# Autodesk Inventor assembly: 垃圾桶
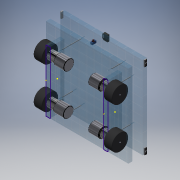
[picture p0: Inventor's stored thumbnail of the model, 180x180]
Saved by Autodesk Inventor 2017 (Build 210142000, 142)
## iProperties
Part Number: 垃圾桶
Material: 常规
Document SubType Name: Assembly
Designer: PANDA
Author: PANDA
## Documents named in this file (9)
- D:\PANDA\Study\VG100\P2\草图\垃圾桶底座.iam
- D:\PANDA\Study\VG100\P2\草图\垃圾桶底板.ipt
- D:\PANDA\Study\VG100\P2\草图\圆柱.ipt
- D:\PANDA\Study\VG100\P2\草图\马达安装板.ipt
- D:\PANDA\Study\VG100\P2\草图\轮子.ipt
- D:\PANDA\Study\VG100\P2\草图\马达.ipt
- D:\PANDA\Study\VG100\P2\草图\红外.ipt
- D:\PANDA\Study\VG100\P2\草图\红外测距.ipt
- D:\PANDA\Study\VG100\P2\草图\姿态传感器.ipt
## Components (26 placed, 8 different names)
1. 垃圾桶底板:1 — 旋转:9, 旋转:10, 旋转:15, 旋转:16, 刚性:2, 刚性:3, 刚性:4, 刚性:5, 刚性:6
2. 圆柱:1 — 旋转:9
3. 圆柱:2 — 旋转:10, 旋转:23
4. 圆柱:3 — 旋转:19
5. 圆柱:4
6. 圆柱:5 — 旋转:15
7. 圆柱:6 — 旋转:16, 旋转:17, 旋转:18
8. 圆柱:7
9. 圆柱:8 — 旋转:22
10. 垃圾桶底板:2 — 旋转:17, 刚性:1
11. 马达安装板:1 — 旋转:18, 旋转:19, 旋转:20, 旋转:21
12. 轮子:1 — 旋转:21, 旋转:29
13. 轮子:2 — 旋转:20, 旋转:28
14. 马达安装板:2 — 旋转:22, 旋转:23, 旋转:24, 旋转:25
15. 轮子:3 — 旋转:25, 旋转:27
16. 轮子:4 — 旋转:24, 旋转:26
17. 马达:1 — 旋转:26
18. 马达:2 — 旋转:27
19. 马达:3 — 旋转:28
20. 马达:4 — 旋转:29
21. 红外:1 — 刚性:1
22. 红外测距:1 — 刚性:2
23. 红外测距:2 — 刚性:3
24. 红外测距:3 — 刚性:5
25. 红外测距:4 — 刚性:4
26. 姿态传感器:1 — 刚性:6
## Relationships (23: RevoluteJoint 17, WeldJoint 6)
- 旋转:9 [RevoluteJoint]: 垃圾桶底板:1 ↔ 圆柱:1
- 旋转:10 [RevoluteJoint]: 垃圾桶底板:1 ↔ 圆柱:2
- 旋转:15 [RevoluteJoint]: 垃圾桶底板:1 ↔ 圆柱:5
- 旋转:16 [RevoluteJoint]: 垃圾桶底板:1 ↔ 圆柱:6
- 旋转:17 [RevoluteJoint]: 圆柱:6 ↔ 垃圾桶底板:2
- 旋转:18 [RevoluteJoint]: 圆柱:6 ↔ 马达安装板:1
- 旋转:19 [RevoluteJoint]: 圆柱:3 ↔ 马达安装板:1
- 旋转:20 [RevoluteJoint]: 马达安装板:1 ↔ 轮子:2
- 旋转:21 [RevoluteJoint]: 马达安装板:1 ↔ 轮子:1
- 旋转:22 [RevoluteJoint]: 圆柱:8 ↔ 马达安装板:2
- 旋转:23 [RevoluteJoint]: 圆柱:2 ↔ 马达安装板:2
- 旋转:24 [RevoluteJoint]: 马达安装板:2 ↔ 轮子:4
- 旋转:25 [RevoluteJoint]: 马达安装板:2 ↔ 轮子:3
- 旋转:26 [RevoluteJoint]: 轮子:4 ↔ 马达:1
- 旋转:27 [RevoluteJoint]: 轮子:3 ↔ 马达:2
- 旋转:28 [RevoluteJoint]: 轮子:2 ↔ 马达:3
- 旋转:29 [RevoluteJoint]: 轮子:1 ↔ 马达:4
- 刚性:1 [WeldJoint]: 垃圾桶底板:2 ↔ 红外:1
- 刚性:2 [WeldJoint]: 垃圾桶底板:1 ↔ 红外测距:1
- 刚性:3 [WeldJoint]: 垃圾桶底板:1 ↔ 红外测距:2
- 刚性:4 [WeldJoint]: 垃圾桶底板:1 ↔ 红外测距:4
- 刚性:5 [WeldJoint]: 垃圾桶底板:1 ↔ 红外测距:3
- 刚性:6 [WeldJoint]: 垃圾桶底板:1 ↔ 姿态传感器:1
